# Autodesk Inventor assembly: chassis_2-02
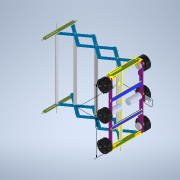
[picture p0: Inventor's stored thumbnail of the model, 180x180]
Saved by Autodesk Inventor 2022 (Build 260153000, 153)
## iProperties
Created: 2023-03-24
Part Number: chassis_2-02
Document SubType Name: Assembly
Designer: Johnny Jou
Author: Johnny Jou
## Documents named in this file (17)
- C:\Users\Johnny Jou\Documents\GitHub\Areo_Rider_Cabin\car\chassis_2.iam
- C:\Users\Johnny Jou\Documents\GitHub\Areo_Rider_Cabin\car\chassis_1_1.ipt
- C:\Users\Johnny Jou\Documents\GitHub\Areo_Rider_Cabin\car\chassis_1_2.ipt
- C:\Users\Johnny Jou\Documents\GitHub\Areo_Rider_Cabin\car\chassis_1_3.ipt
- C:\Users\Johnny Jou\Documents\GitHub\Areo_Rider_Cabin\car\chassis_1_4.ipt
- C:\Users\Johnny Jou\Documents\GitHub\Areo_Rider_Cabin\car\wheel.ipt
- C:\Users\Johnny Jou\Documents\GitHub\Areo_Rider_Cabin\car\wheel_base_cover.ipt
- C:\Users\Johnny Jou\Documents\GitHub\Areo_Rider_Cabin\car\bearing.iam
- C:\Users\Johnny Jou\Documents\GitHub\Areo_Rider_Cabin\car\axle 4_20.ipt
- C:\Users\Johnny Jou\Documents\GitHub\Areo_Rider_Cabin\car\Coupling.ipt
- C:\Users\Johnny Jou\Documents\GitHub\Areo_Rider_Cabin\motor\25GA370.ipt
- C:\Users\Johnny Jou\Documents\GitHub\Areo_Rider_Cabin\car\chassis_1_1\chassis_1_1-01.ipt
- C:\Users\Johnny Jou\Documents\GitHub\Areo_Rider_Cabin\Expansion\gasket.ipt
- C:\Users\Johnny Jou\Documents\GitHub\Areo_Rider_Cabin\Expansion\link_2022.ipt
- C:\Users\Johnny Jou\Documents\GitHub\Areo_Rider_Cabin\Expansion\rod_2.ipt
- C:\Users\Johnny Jou\Documents\GitHub\Areo_Rider_Cabin\car\chassis_1_2_up.ipt
- C:\Users\Johnny Jou\Documents\GitHub\Areo_Rider_Cabin\Expansion\rod_3.ipt
## Components (61 placed, 16 different names)
1. chassis_1_1:1 — 貼合:1, 齊平:2, 貼合:6, 齊平:5, 貼合:7, 貼合:8, 齊平:6, 貼合:9, 齊平:8, 齊平:12, 貼合:40, 貼合:41, 貼合:42, 貼合:43, 貼合:44, 貼合:45, 貼合:66, 貼合:67, 貼合:68, 齊平:31, 貼合:80, 上升與下降
2. chassis_1_2:1 — 貼合:1, 齊平:2, 貼合:10, 齊平:7, 齊平:10, 插入:9, 貼合:86, 貼合:93
3. chassis_1_3:1 — 貼合:6, 齊平:5, 貼合:7, 齊平:25
4. chassis_1_3:2 — 貼合:8, 齊平:6, 貼合:9, 貼合:78, 角度:1
5. chassis_1_4:1 — 貼合:10, 齊平:7, 齊平:8, 齊平:11
6. chassis_1_4:2 — 齊平:10, 齊平:11, 齊平:28
7. chassis_1_4:3 — 齊平:12, 齊平:14, 齊平:32
8. chassis_1_4:4 — 齊平:14, 齊平:27, 貼合:91, 齊平:33
9. wheel:1 — 貼合:16, 貼合:17, 貼合:18
10. wheel_base_cover:1 — 貼合:12, 齊平:17, 貼合:15, 貼合:41, 貼合:42
11. 軸承:1 [sub-assembly] — 貼合:12, 齊平:17, 貼合:13, 齊平:18
12. axle 4_20:1 — 貼合:13, 齊平:18, 貼合:14, 貼合:40
13. Coupling:1 — 貼合:14, 貼合:15, 貼合:16, 貼合:17, 貼合:18
14. wheel:2
15. wheel_base_cover:2 — 貼合:43, 貼合:44, 貼合:45
16. 軸承:2 [sub-assembly]
17. axle 4_20:2
18. Coupling:2
19. wheel:3
20. wheel_base_cover:3 — 貼合:71, 貼合:72, 貼合:77
21. 軸承:3 [sub-assembly]
22. axle 4_20:3
23. Coupling:3
24. wheel:4
25. wheel_base_cover:4 — 貼合:69, 貼合:70, 貼合:76
26. 軸承:4 [sub-assembly]
27. axle 4_20:4
28. Coupling:4
29. wheel:5
30. Coupling:5 — 貼合:59, 貼合:60
31. 25GA370:1 — 貼合:59, 貼合:60, 貼合:66, 貼合:67, 貼合:68
32. wheel:6
33. Coupling:6
34. 25GA370:2 — 貼合:73, 貼合:74, 貼合:75
35. chassis_1_1-01:2 — 貼合:69, 貼合:70, 貼合:71, 貼合:72, 貼合:73, 貼合:74, 貼合:75, 貼合:76, 貼合:77, 貼合:78, 齊平:25, 齊平:27, 齊平:28, 齊平:30, 貼合:86, 貼合:92, 貼合:93
36. link_2022:1 — 插入:8, 貼合:97, 貼合:100
37. link_2022:2 — 貼合:79, 插入:28
38. link_2022:3
39. link_2022:4 — 貼合:96, 貼合:99
40. link_2022:5 — 插入:23
41. link_2022:6 — 插入:25, 貼合:95, 貼合:98
42. gasket:1 — 插入:8, 插入:9
43. rod_2:1 — 貼合:79, 貼合:81, 貼合:82, 角度:1, 貼合:83, 上升與下降
44. chassis_1_2:2 — 齊平:30, 齊平:31, 貼合:80, 齊平:32, 插入:17, 貼合:83, 貼合:91, 齊平:33, 貼合:92
45. link_2022:7 — 插入:17
46. link_2022:8 — 貼合:81, 貼合:82, 插入:27
47. link_2022:9
48. link_2022:10
49. link_2022:11 — 插入:21
50. link_2022:12 — 貼合:88, 插入:26
51. chassis_1_2_up:1 — 插入:23
52. chassis_1_2_up:2 — 角度:2, 貼合:89, 插入:22
53. rod_3:1 — 貼合:88, 角度:2, 貼合:89, 貼合:94
54. gasket:3 — 插入:21, 插入:22
55. gasket:5 — 插入:25
56. gasket:6 — 插入:26, 貼合:94
57. gasket:7 — 插入:27
58. gasket:8 — 插入:28
59. rod_3:2 — 貼合:95, 貼合:98
60. rod_3:3 — 貼合:96, 貼合:99
61. rod_3:4 — 貼合:97, 貼合:100
## Relationships (132: Mate 82, Flush 24, Insert 24, Angle 2)
- 貼合:1 [Mate]: chassis_1_1:1 ↔ chassis_1_2:1
- 齊平:2 [Flush]: chassis_1_1:1 ↔ chassis_1_2:1
- 貼合:6 [Mate]: chassis_1_1:1 ↔ chassis_1_3:1
- 齊平:5 [Flush]: chassis_1_1:1 ↔ chassis_1_3:1
- 貼合:7 [Mate]: chassis_1_1:1 ↔ chassis_1_3:1
- 貼合:8 [Mate]: chassis_1_1:1 ↔ chassis_1_3:2
- 齊平:6 [Flush]: chassis_1_1:1 ↔ chassis_1_3:2
- 貼合:9 [Mate]: chassis_1_1:1 ↔ chassis_1_3:2
- 貼合:10 [Mate]: chassis_1_2:1 ↔ chassis_1_4:1
- 齊平:7 [Flush]: chassis_1_2:1 ↔ chassis_1_4:1
- 齊平:8 [Flush]: chassis_1_1:1 ↔ chassis_1_4:1
- 齊平:10 [Flush]: chassis_1_2:1 ↔ chassis_1_4:2
- 齊平:11 [Flush]: chassis_1_4:1 ↔ chassis_1_4:2
- 齊平:12 [Flush]: chassis_1_1:1 ↔ chassis_1_4:3
- 齊平:14 [Flush]: chassis_1_4:3 ↔ chassis_1_4:4
- 貼合:12 [Mate]: wheel_base_cover:1 ↔ 軸承:1
- 齊平:17 [Flush]: wheel_base_cover:1 ↔ 軸承:1
- 貼合:13 [Mate]: 軸承:1 ↔ axle 4_20:1
- 齊平:18 [Flush]: 軸承:1 ↔ axle 4_20:1
- 貼合:14 [Mate]: axle 4_20:1 ↔ Coupling:1
- 貼合:15 [Mate] (6 mm): wheel_base_cover:1 ↔ Coupling:1
- 貼合:16 [Mate]: wheel:1 ↔ Coupling:1
- 貼合:17 [Mate]: wheel:1 ↔ Coupling:1
- 貼合:18 [Mate]: wheel:1 ↔ Coupling:1
- [Mate]: wheel_base_cover:2 ↔ 軸承:2
- [Flush]: wheel_base_cover:2 ↔ 軸承:2
- [Mate]: 軸承:2 ↔ axle 4_20:2
- [Flush]: 軸承:2 ↔ axle 4_20:2
- [Mate]: axle 4_20:2 ↔ Coupling:2
- [Mate] (6 mm): wheel_base_cover:2 ↔ Coupling:2
- [Mate]: wheel:2 ↔ Coupling:2
- [Mate]: wheel:2 ↔ Coupling:2
- [Mate]: wheel:2 ↔ Coupling:2
- [Mate]: wheel_base_cover:3 ↔ 軸承:3
- [Flush]: wheel_base_cover:3 ↔ 軸承:3
- [Mate]: 軸承:3 ↔ axle 4_20:3
- [Flush]: 軸承:3 ↔ axle 4_20:3
- [Mate]: axle 4_20:3 ↔ Coupling:3
- [Mate] (6 mm): wheel_base_cover:3 ↔ Coupling:3
- [Mate]: wheel:3 ↔ Coupling:3
- [Mate]: wheel:3 ↔ Coupling:3
- [Mate]: wheel:3 ↔ Coupling:3
- [Mate]: wheel_base_cover:4 ↔ 軸承:4
- [Flush]: wheel_base_cover:4 ↔ 軸承:4
- [Mate]: 軸承:4 ↔ axle 4_20:4
- [Flush]: 軸承:4 ↔ axle 4_20:4
- [Mate]: axle 4_20:4 ↔ Coupling:4
- [Mate] (6 mm): wheel_base_cover:4 ↔ Coupling:4
- [Mate]: wheel:4 ↔ Coupling:4
- [Mate]: wheel:4 ↔ Coupling:4
- [Mate]: wheel:4 ↔ Coupling:4
- 貼合:40 [Mate]: chassis_1_1:1 ↔ axle 4_20:1
- 貼合:41 [Mate]: chassis_1_1:1 ↔ wheel_base_cover:1
- 貼合:42 [Mate]: chassis_1_1:1 ↔ wheel_base_cover:1
- 貼合:43 [Mate]: chassis_1_1:1 ↔ wheel_base_cover:2
- 貼合:44 [Mate]: chassis_1_1:1 ↔ wheel_base_cover:2
- 貼合:45 [Mate]: chassis_1_1:1 ↔ wheel_base_cover:2
- [Mate]: wheel:5 ↔ Coupling:5
- [Mate]: wheel:5 ↔ Coupling:5
- [Mate]: wheel:5 ↔ Coupling:5
- 貼合:59 [Mate]: Coupling:5 ↔ 25GA370:1
- 貼合:60 [Mate] (6 mm): Coupling:5 ↔ 25GA370:1
- [Mate]: wheel:6 ↔ Coupling:6
- [Mate]: wheel:6 ↔ Coupling:6
- [Mate]: wheel:6 ↔ Coupling:6
- [Mate]: Coupling:6 ↔ 25GA370:2
- [Mate] (6 mm): Coupling:6 ↔ 25GA370:2
- 貼合:66 [Mate]: chassis_1_1:1 ↔ 25GA370:1
- 貼合:67 [Mate]: chassis_1_1:1 ↔ 25GA370:1
- 貼合:68 [Mate]: chassis_1_1:1 ↔ 25GA370:1
- 貼合:69 [Mate]: wheel_base_cover:4 ↔ chassis_1_1-01:2
- 貼合:70 [Mate]: wheel_base_cover:4 ↔ chassis_1_1-01:2
- 貼合:71 [Mate]: wheel_base_cover:3 ↔ chassis_1_1-01:2
- 貼合:72 [Mate]: wheel_base_cover:3 ↔ chassis_1_1-01:2
- 貼合:73 [Mate]: 25GA370:2 ↔ chassis_1_1-01:2
- 貼合:74 [Mate]: 25GA370:2 ↔ chassis_1_1-01:2
- 貼合:75 [Mate]: 25GA370:2 ↔ chassis_1_1-01:2
- 貼合:76 [Mate]: wheel_base_cover:4 ↔ chassis_1_1-01:2
- 貼合:77 [Mate]: wheel_base_cover:3 ↔ chassis_1_1-01:2
- 貼合:78 [Mate]: chassis_1_3:2 ↔ chassis_1_1-01:2
- 齊平:25 [Flush]: chassis_1_3:1 ↔ chassis_1_1-01:2
- 齊平:27 [Flush]: chassis_1_4:4 ↔ chassis_1_1-01:2
- 齊平:28 [Flush]: chassis_1_4:2 ↔ chassis_1_1-01:2
- [Insert]: link_2022:1 ↔ link_2022:2
- [Insert]: link_2022:1 ↔ link_2022:3
- [Insert]: link_2022:2 ↔ link_2022:4
- [Insert]: link_2022:3 ↔ link_2022:4
- [Insert]: link_2022:5 ↔ link_2022:6
- [Insert]: link_2022:4 ↔ link_2022:5
- [Insert]: link_2022:3 ↔ link_2022:6
- 插入:8 [Insert]: link_2022:1 ↔ gasket:1
- 插入:9 [Insert]: chassis_1_2:1 ↔ gasket:1
- 貼合:79 [Mate]: link_2022:2 ↔ rod_2:1
- 齊平:30 [Flush]: chassis_1_1-01:2 ↔ chassis_1_2:2
- 齊平:31 [Flush]: chassis_1_1:1 ↔ chassis_1_2:2
- 貼合:80 [Mate]: chassis_1_1:1 ↔ chassis_1_2:2
- 齊平:32 [Flush]: chassis_1_4:3 ↔ chassis_1_2:2
- [Insert]: link_2022:7 ↔ link_2022:8
- [Insert]: link_2022:7 ↔ link_2022:9
- [Insert]: link_2022:8 ↔ link_2022:10
- [Insert]: link_2022:9 ↔ link_2022:10
- [Insert]: link_2022:11 ↔ link_2022:12
- [Insert]: link_2022:10 ↔ link_2022:11
- [Insert]: link_2022:9 ↔ link_2022:12
- 插入:17 [Insert]: chassis_1_2:2 ↔ link_2022:7
- 貼合:81 [Mate]: rod_2:1 ↔ link_2022:8
- 貼合:82 [Mate]: rod_2:1 ↔ link_2022:8
- 角度:1 [Angle] (180 deg): chassis_1_3:2 ↔ rod_2:1
- 貼合:83 [Mate]: rod_2:1 ↔ chassis_1_2:2
- 貼合:86 [Mate]: chassis_1_2:1 ↔ chassis_1_1-01:2
- 上升與下降 [Mate] (75 mm): chassis_1_1:1 ↔ rod_2:1
- 貼合:88 [Mate]: link_2022:12 ↔ rod_3:1
- 角度:2 [Angle] (0 deg): chassis_1_2_up:2 ↔ rod_3:1
- 貼合:89 [Mate]: chassis_1_2_up:2 ↔ rod_3:1
- 插入:21 [Insert]: link_2022:11 ↔ gasket:3
- 插入:22 [Insert]: chassis_1_2_up:2 ↔ gasket:3
- 插入:23 [Insert]: link_2022:5 ↔ chassis_1_2_up:1
- 貼合:91 [Mate]: chassis_1_4:4 ↔ chassis_1_2:2
- 齊平:33 [Flush]: chassis_1_4:4 ↔ chassis_1_2:2
- 貼合:92 [Mate]: chassis_1_1-01:2 ↔ chassis_1_2:2
- 貼合:93 [Mate]: chassis_1_2:1 ↔ chassis_1_1-01:2
- 插入:25 [Insert]: link_2022:6 ↔ gasket:5
- 插入:26 [Insert]: link_2022:12 ↔ gasket:6
- 貼合:94 [Mate]: rod_3:1 ↔ gasket:6
- 插入:27 [Insert]: link_2022:8 ↔ gasket:7
- 插入:28 [Insert]: link_2022:2 ↔ gasket:8
- 貼合:95 [Mate]: link_2022:6 ↔ rod_3:2
- 貼合:96 [Mate]: link_2022:4 ↔ rod_3:3
- 貼合:97 [Mate]: link_2022:1 ↔ rod_3:4
- 貼合:98 [Mate]: link_2022:6 ↔ rod_3:2
- 貼合:99 [Mate]: link_2022:4 ↔ rod_3:3
- 貼合:100 [Mate]: link_2022:1 ↔ rod_3:4
## Named parameters: d118_d109 = 0 mm, d119_d110 = 0 mm, d120_d111 = 0 mm, d121_d112 = 0 mm, d122_d113 = 0 mm, d123_d114 = 6 mm, d124_d115 = 0 mm, d125_d116 = 0 mm, d126_d117 = 0 mm, d127_d109 = 0 mm, d128_d110 = 0 mm, d129_d111 = 0 mm, d130_d112 = 0 mm, d131_d113 = 0 mm, d132_d114 = 6 mm, d133_d115 = 0 mm, d134_d116 = 0 mm, d135_d117 = 0 mm, d136_d109 = 0 mm, d137_d110 = 0 mm, d138_d111 = 0 mm, d139_d112 = 0 mm, d140_d113 = 0 mm, d141_d114 = 6 mm, d142_d115 = 0 mm, d143_d116 = 0 mm, d144_d117 = 0 mm, d163_d115 = 0 mm, d164_d116 = 0 mm, d165_d117 = 0 mm, d168_d163_d115 = 0 mm, d169_d164_d116 = 0 mm, d170_d165_d117 = 0 mm, d171_d166 = 0 mm, d172_d167 = 6 mm, d4_d3 = 0 mm, d215_d0 = 0 mm, d216_d1 = 0 mm, d217_d2 = 0 mm, d218_d3 = 0 mm, d219_d4_d3 = 0 mm, d220_d5 = 0 mm, d221_d6 = 0 mm
